# Autodesk Inventor assembly: 20 pixel strip
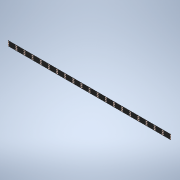
[picture p0: Inventor's stored thumbnail of the model, 180x180]
Saved by Autodesk Inventor 2020 (Build 240168000, 168)
## iProperties
Created: 2021-03-06
Part Number: 20 pixel strip
Document SubType Name: Assembly
Designer: Harry
Author: Harry
## Documents named in this file (2)
- C:\Users\Harry\Documents\hacktheburgh\octocatch\cad\20 pixel strip.iam
- C:\Users\Harry\Documents\hacktheburgh\octocatch\cad\WS2812B Black 60leds_m v7.ipt
## Components (20 placed, 1 different names)
1. WS2812B Black 60leds_m v7:1
2. WS2812B Black 60leds_m v7:2
3. WS2812B Black 60leds_m v7:3
4. WS2812B Black 60leds_m v7:4
5. WS2812B Black 60leds_m v7:5
6. WS2812B Black 60leds_m v7:6
7. WS2812B Black 60leds_m v7:7
8. WS2812B Black 60leds_m v7:8
9. WS2812B Black 60leds_m v7:9
10. WS2812B Black 60leds_m v7:10
11. WS2812B Black 60leds_m v7:11
12. WS2812B Black 60leds_m v7:12
13. WS2812B Black 60leds_m v7:13
14. WS2812B Black 60leds_m v7:14
15. WS2812B Black 60leds_m v7:15
16. WS2812B Black 60leds_m v7:16
17. WS2812B Black 60leds_m v7:17
18. WS2812B Black 60leds_m v7:18
19. WS2812B Black 60leds_m v7:19
20. WS2812B Black 60leds_m v7:20
## Component patterns: (20 elements, first: WS2812B Black 60leds_m v7:1)
